# Autodesk Inventor assembly: RightLowerLimbBlock
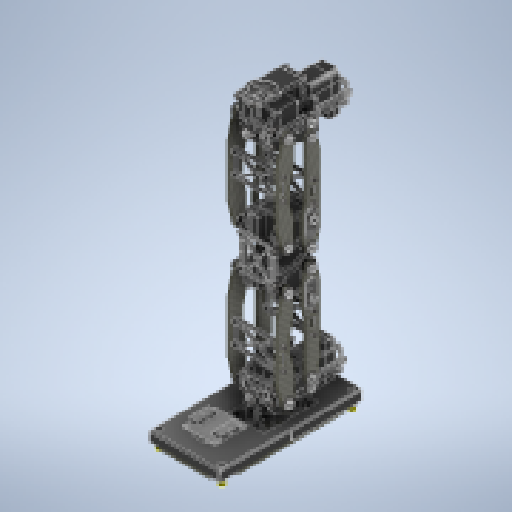
[picture p0: Inventor's stored thumbnail of the model, 512x512]
Saved by Autodesk Inventor 2024.2 (Build 282272000, 272)
## iProperties
Created: 2024-01-05
Part Number: RightLowerLimbBlock
Document SubType Name: Assembly
Designer: Masato Kubotera
Mass: 1508.63 g
Surface Area: 4073.7 cm^2
Volume: 695.465 cm^3
Density: 2.16924 g/cm^3
Author: Masato Kubotera
## Documents named in this file (18)
- D:\OneDrive - Chiba Institute of Technology\CIT Brains\RoboCup2024\Mechanic\SUSTAINA-OP2-DEV\NativeFiles\Boby\LowerLimb\RightLowerLimbBlock.iam
- D:\OneDrive - Chiba Institute of Technology\CIT Brains\RoboCup2024\Mechanic\SUSTAINA-OP2-DEV\NativeFiles\Boby\LowerLimb\Hips\HipUnit.iam
- D:\OneDrive - Chiba Institute of Technology\CIT Brains\RoboCup2024\Mechanic\SUSTAINA-OP2-DEV\NativeFiles\Boby\LowerLimb\Legs\Links\LegUpperFrontLinkUnit.iam
- D:\OneDrive - Chiba Institute of Technology\CIT Brains\RoboCup2024\Mechanic\SUSTAINA-OP2-DEV\NativeFiles\Boby\LowerLimb\Legs\Knees\KneeUnit.iam
- D:\OneDrive - Chiba Institute of Technology\CIT Brains\RoboCup2024\Mechanic\SUSTAINA-OP2-DEV\NativeFiles\Boby\LowerLimb\Legs\LegBases\UpperLegBaseRollCrankUnit.iam
- D:\OneDrive - Chiba Institute of Technology\CIT Brains\RoboCup2024\Mechanic\SUSTAINA-OP2-DEV\NativeFiles\Boby\LowerLimb\Legs\LegBases\LowerLegBaseRollCrankUnit.iam
- D:\OneDrive - Chiba Institute of Technology\CIT Brains\RoboCup2024\Mechanic\SUSTAINA-OP2-DEV\NativeFiles\Boby\LowerLimb\Feet\RightFootUnit.iam
- D:\OneDrive - Chiba Institute of Technology\CIT Brains\RoboCup2024\Mechanic\SUSTAINA-OP2-DEV\NativeFiles\Boby\LowerLimb\Legs\Knees\KneeBackSlashCutCrankUnit.iam
- D:\OneDrive - Chiba Institute of Technology\CIT Brains\RoboCup2024\Mechanic\SUSTAINA-OP2-DEV\NativeFiles\Boby\LowerLimb\Legs\Knees\KneeSlashCutCrankUnit.iam
- D:\OneDrive - Chiba Institute of Technology\CIT Brains\RoboCup2024\Mechanic\SUSTAINA-OP2-DEV\NativeFiles\Boby\LowerLimb\Legs\LegBases\LegBaseSlashCutCrankUnit.iam
- D:\OneDrive - Chiba Institute of Technology\CIT Brains\RoboCup2024\Mechanic\SUSTAINA-OP2-DEV\NativeFiles\Boby\LowerLimb\Legs\LegBases\LegBaseBackSlashCutCrankUnit.iam
- D:\OneDrive - Chiba Institute of Technology\CIT Brains\RoboCup2024\Mechanic\SUSTAINA-OP2-DEV\NativeFiles\Boby\LowerLimb\Legs\LegBases\LegAnkleUnit_MIR.iam
- D:\OneDrive - Chiba Institute of Technology\CIT Brains\RoboCup2024\Mechanic\SUSTAINA-OP2-DEV\NativeFiles\Boby\LowerLimb\Legs\LegBases\LegGroinUnit_MIR.iam
- D:\OneDrive - Chiba Institute of Technology\CIT Brains\RoboCup2024\Mechanic\SUSTAINA-OP2-DEV\NativeFiles\Boby\LowerLimb\Legs\Links\LegUpperBackLinkUnit_MIR.iam
- D:\OneDrive - Chiba Institute of Technology\CIT Brains\RoboCup2024\Mechanic\SUSTAINA-OP2-DEV\NativeFiles\Boby\LowerLimb\Legs\Links\LegLowerBackLinkUnit_MIR.iam
- D:\OneDrive - Chiba Institute of Technology\CIT Brains\RoboCup2024\Mechanic\SUSTAINA-OP2-DEV\NativeFiles\Boby\LowerLimb\Legs\Links\LegLowerFrontLinkUnit.iam
- D:\OneDrive - Chiba Institute of Technology\CIT Brains\RoboCup2024\Mechanic\SUSTAINA-OP2-DEV\NativeFiles\Boby\LowerLimb\Legs\Links\ParallelLinksDriveUpperUnit_MIR.iam
- D:\OneDrive - Chiba Institute of Technology\CIT Brains\RoboCup2024\Mechanic\SUSTAINA-OP2-DEV\NativeFiles\Boby\LowerLimb\Legs\Links\ParallelLinksDriveLowerUnit_MIR.iam
## Components (17 placed, 17 different names)
1. HipUnit:1 [sub-assembly] — Hip-Yaw, Mate:1, Flush:1, Insert:1, Insert:2
2. LegGroinUnit_MIR:1 [sub-assembly] — Insert:1, Insert:2, Hip-Roll, Insert:3, [Auto]Hip-Roll-Crank, Insert:4, Insert:5, Hip-Pitch, Insert:6, [Auto]Hip-Pitch-Crank
3. UpperLegBaseRollCrankUnit:1 [sub-assembly] — Insert:3, [Auto]Hip-Roll-Crank
4. ParallelLinksDriveUpperUnit_MIR:1 [sub-assembly] — Insert:4, Insert:5, Hip-Pitch, Insert:7, Insert:8, Insert:9, Insert:10
5. LegBaseSlashCutCrankUnit:1 [sub-assembly] — Insert:6, [Auto]Hip-Pitch-Crank
6. LegUpperBackLinkUnit_MIR:1 [sub-assembly] — Insert:9, Insert:10, Insert:13, Insert:14, UpperKnee-Pitch
7. LegUpperFrontLinkUnit:1 [sub-assembly] — Insert:7, Insert:8, Insert:11, Insert:12
8. KneeUnit:1 [sub-assembly] — Insert:11, Insert:12, Insert:13, Insert:14, UpperKnee-Pitch, LowerKnee-Pitch, Insert:15, [Auto]UpperKnee-Pitch-Crank, [Auto]LowerKnee-Pitch-Crank, Insert:16, Insert:17, Insert:18, Insert:19, Insert:20
9. KneeSlashCutCrankUnit:1 [sub-assembly] — Insert:15, [Auto]UpperKnee-Pitch-Crank
10. LegLowerBackLinkUnit_MIR:1 [sub-assembly] — Insert:18, Insert:19, Insert:23, Insert:24, LowerKnee-Pitch
11. LegLowerFrontLinkUnit:1 [sub-assembly] — Insert:16, Insert:17, Insert:21, Insert:22
12. KneeBackSlashCutCrankUnit:1 [sub-assembly] — Insert:20, [Auto]LowerKnee-Pitch-Crank
13. ParallelLinksDriveLowerUnit_MIR:1 [sub-assembly] — Insert:21, Insert:22, Insert:23, Insert:24, Insert:25, Insert:26, Ankle-Pitch
14. LegAnkleUnit_MIR:1 [sub-assembly] — Insert:25, Insert:26, Ankle-Pitch, Insert:27, [Auto]Ankle-Pitch-Crank, Insert:29, Insert:30, Insert:31
15. LegBaseBackSlashCutCrankUnit:1 [sub-assembly] — Insert:27, [Auto]Ankle-Pitch-Crank, Ankle-Roll, [Auto]Ankle-Roll-Crank
16. LowerLegBaseRollCrankUnit:1 [sub-assembly] — Insert:30, [Auto]Ankle-Roll-Crank
17. RightFootUnit:1 [sub-assembly] — Insert:29, Ankle-Roll, Insert:31
## Relationships (45: Insert 30, Angle 13, Mate 1, Flush 1)
- Hip-Yaw [Angle] (0 deg): HipUnit:1
- Hip-Roll [Angle] (0 deg): LegGroinUnit_MIR:1
- Hip-Pitch [Angle] (0 deg): LegGroinUnit_MIR:1 ↔ ParallelLinksDriveUpperUnit_MIR:1
- UpperKnee-Pitch [Angle] (180 deg): LegUpperBackLinkUnit_MIR:1 ↔ KneeUnit:1
- LowerKnee-Pitch [Angle] (180 deg): KneeUnit:1 ↔ LegLowerBackLinkUnit_MIR:1
- Ankle-Pitch [Angle] (180 deg): ParallelLinksDriveLowerUnit_MIR:1 ↔ LegAnkleUnit_MIR:1
- Ankle-Roll [Angle] (180 deg): LegBaseBackSlashCutCrankUnit:1 ↔ RightFootUnit:1
- [Auto]Hip-Roll-Crank [Angle] (0 deg): LegGroinUnit_MIR:1 ↔ UpperLegBaseRollCrankUnit:1
- [Auto]Hip-Pitch-Crank [Angle] (0 deg): LegGroinUnit_MIR:1 ↔ LegBaseSlashCutCrankUnit:1
- [Auto]UpperKnee-Pitch-Crank [Angle] (-360 deg): KneeUnit:1 ↔ KneeSlashCutCrankUnit:1
- [Auto]LowerKnee-Pitch-Crank [Angle] (-360 deg): KneeUnit:1 ↔ KneeBackSlashCutCrankUnit:1
- [Auto]Ankle-Pitch-Crank [Angle] (-180 deg): LegAnkleUnit_MIR:1 ↔ LegBaseBackSlashCutCrankUnit:1
- [Auto]Ankle-Roll-Crank [Angle] (180 deg): LegBaseBackSlashCutCrankUnit:1 ↔ LowerLegBaseRollCrankUnit:1
- Mate:1: HipUnit:1
- Flush:1: HipUnit:1
- Insert:1: HipUnit:1 ↔ LegGroinUnit_MIR:1
- Insert:2: HipUnit:1 ↔ LegGroinUnit_MIR:1
- Insert:3: LegGroinUnit_MIR:1 ↔ UpperLegBaseRollCrankUnit:1
- Insert:4: LegGroinUnit_MIR:1 ↔ ParallelLinksDriveUpperUnit_MIR:1
- Insert:5: LegGroinUnit_MIR:1 ↔ ParallelLinksDriveUpperUnit_MIR:1
- Insert:6: LegGroinUnit_MIR:1 ↔ LegBaseSlashCutCrankUnit:1
- Insert:7: ParallelLinksDriveUpperUnit_MIR:1 ↔ LegUpperFrontLinkUnit:1
- Insert:8: ParallelLinksDriveUpperUnit_MIR:1 ↔ LegUpperFrontLinkUnit:1
- Insert:9: ParallelLinksDriveUpperUnit_MIR:1 ↔ LegUpperBackLinkUnit_MIR:1
- Insert:10: ParallelLinksDriveUpperUnit_MIR:1 ↔ LegUpperBackLinkUnit_MIR:1
- Insert:11: LegUpperFrontLinkUnit:1 ↔ KneeUnit:1
- Insert:12: LegUpperFrontLinkUnit:1 ↔ KneeUnit:1
- Insert:13: LegUpperBackLinkUnit_MIR:1 ↔ KneeUnit:1
- Insert:14: LegUpperBackLinkUnit_MIR:1 ↔ KneeUnit:1
- Insert:15: KneeUnit:1 ↔ KneeSlashCutCrankUnit:1
- Insert:16: KneeUnit:1 ↔ LegLowerFrontLinkUnit:1
- Insert:17: KneeUnit:1 ↔ LegLowerFrontLinkUnit:1
- Insert:18: KneeUnit:1 ↔ LegLowerBackLinkUnit_MIR:1
- Insert:19: KneeUnit:1 ↔ LegLowerBackLinkUnit_MIR:1
- Insert:20: KneeUnit:1 ↔ KneeBackSlashCutCrankUnit:1
- Insert:21: LegLowerFrontLinkUnit:1 ↔ ParallelLinksDriveLowerUnit_MIR:1
- Insert:22: LegLowerFrontLinkUnit:1 ↔ ParallelLinksDriveLowerUnit_MIR:1
- Insert:23: LegLowerBackLinkUnit_MIR:1 ↔ ParallelLinksDriveLowerUnit_MIR:1
- Insert:24: LegLowerBackLinkUnit_MIR:1 ↔ ParallelLinksDriveLowerUnit_MIR:1
- Insert:25: ParallelLinksDriveLowerUnit_MIR:1 ↔ LegAnkleUnit_MIR:1
- Insert:26: ParallelLinksDriveLowerUnit_MIR:1 ↔ LegAnkleUnit_MIR:1
- Insert:27: LegAnkleUnit_MIR:1 ↔ LegBaseBackSlashCutCrankUnit:1
- Insert:29: LegAnkleUnit_MIR:1 ↔ RightFootUnit:1
- Insert:30: LegAnkleUnit_MIR:1 ↔ LowerLegBaseRollCrankUnit:1
- Insert:31: LegAnkleUnit_MIR:1 ↔ RightFootUnit:1
## Named parameters: HipYaw = 0 deg, HipRoll = 0 deg, HipRollCrank = 0 deg, HipPitch = 0 deg, HipPitchCrank = 0 deg, UpperKneePitch = 180 deg, UpperKneePitchCrank = -360 deg, LowerKneePitch = 180 deg, LowerKneePitchCrank = -360 deg, AnklePitch = 180 deg, AnklePitchCrank = -180 deg, AnkleRoll = 180 deg, AnkleRollCrank = 180 deg
